# Autodesk Inventor assembly: gearbox
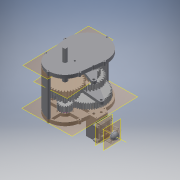
[picture p0: Inventor's stored thumbnail of the model, 180x180]
Saved by Autodesk Inventor 2017 (Build 210142000, 142)
## iProperties
Created: 2018-04-16
Part Number: gearbox
Document SubType Name: Assembly
Designer: RKL
Author: RKL
## Documents named in this file (22)
- C:\Users\RKL\Documents\GitHub\Vane_motor_steam_engine\rotary die grinder engine\transmission\gearbox.iam
- C:\Users\RKL\Documents\GitHub\Vane_motor_steam_engine\rotary die grinder engine\transmission\gearbox\Design Accelerator\Spur Gears1.iam
- C:\Users\RKL\Documents\GitHub\Vane_motor_steam_engine\rotary die grinder engine\transmission\square shaft 1.ipt
- C:\Users\RKL\Documents\GitHub\Vane_motor_steam_engine\rotary die grinder engine\transmission\square bearing adapter.ipt
- C:\Users\RKL\Documents\GitHub\Vane_motor_steam_engine\rotary die grinder engine\transmission\6003 bearing.ipt
- C:\Users\RKL\Documents\GitHub\Vane_motor_steam_engine\rotary die grinder engine\transmission\dog clutch.ipt
- C:\Users\RKL\Documents\GitHub\Vane_motor_steam_engine\rotary die grinder engine\transmission\gearbox\Design Accelerator\Spur Gears2.iam
- C:\Users\RKL\Documents\GitHub\Vane_motor_steam_engine\rotary die grinder engine\transmission\gearbox\Design Accelerator\Spur Gears3.iam
- C:\Users\RKL\Documents\GitHub\Vane_motor_steam_engine\rotary die grinder engine\transmission\gearbox\Design Accelerator\Spur Gears4.iam
- C:\Users\RKL\Documents\GitHub\Vane_motor_steam_engine\rotary die grinder engine\transmission\gearbox\Design Accelerator\Spur Gears5.iam
- C:\Users\RKL\Documents\GitHub\Vane_motor_steam_engine\rotary die grinder engine\transmission\case part 1.ipt
- C:\Users\RKL\Documents\GitHub\Vane_motor_steam_engine\rotary die grinder engine\transmission\fork.ipt
- C:\Users\RKL\Documents\GitHub\Vane_motor_steam_engine\rotary die grinder engine\transmission\shifter box 1.ipt
- C:\Users\RKL\Documents\GitHub\Vane_motor_steam_engine\rotary die grinder engine\transmission\short selector.ipt
- C:\Users\RKL\Documents\GitHub\Vane_motor_steam_engine\rotary die grinder engine\transmission\long selector.ipt
- C:\Users\RKL\Documents\GitHub\Vane_motor_steam_engine\rotary die grinder engine\transmission\shifter cover.ipt
- C:\Users\RKL\Documents\GitHub\Vane_motor_steam_engine\rotary die grinder engine\transmission\shifter cover_MIR.ipt
- C:\Users\RKL\Documents\GitHub\Vane_motor_steam_engine\rotary die grinder engine\transmission\shifter ball.ipt
- C:\Users\RKL\Documents\GitHub\Vane_motor_steam_engine\rotary die grinder engine\transmission\case bottom half.ipt
- C:\Users\RKL\Documents\GitHub\Vane_motor_steam_engine\rotary die grinder engine\transmission\case part 2.ipt
- C:\Users\RKL\Documents\GitHub\Vane_motor_steam_engine\rotary die grinder engine\transmission\case top half.ipt
- C:\Users\RKL\Documents\GitHub\Vane_motor_steam_engine\rotary die grinder engine\transmission\gearbox\gear spacer 1.ipt
## Components (37 placed, 17 different names)
1. Spur Gears:1 [sub-assembly] — Mate:1, Mate:2, Mate:3, Mate:7, Mate:8, Mate:35, Mate:36, Mate:60, Flush:5, Flush:6, Mate:77
2. square shaft 1:1 — Mate:7, Mate:8, Mate:22, Mate:23, Mate:31, Mate:32, Mate:49, Mate:50, Flush:3, Mate:53, Mate:54, Mate:91
3. square shaft 1:2 — Mate:5, Mate:6, Mate:9, Mate:10, Mate:20, Mate:21, Mate:29, Mate:30, Mate:33, Mate:34, Mate:38, Mate:39, Flush:1, Mate:47, Mate:48, Mate:56, Mate:57, Mate:92
4. square bearing adapter:1 — Mate:3, Mate:4, Mate:5, Mate:6
5. 6003 bearing:1 — Mate:1, Mate:2, Mate:4
6. dog clutch:1 — Mate:9, Mate:10, Mate:67, Mate:68
7. Spur Gears:2 [sub-assembly] — Mate:16, Mate:17, Mate:18, Mate:22, Mate:23, Mate:28, Mate:77
8. 6003 bearing:2 — Mate:16, Mate:17, Mate:19
9. square bearing adapter:2 — Mate:18, Mate:19, Mate:20, Mate:21
10. Spur Gears:3 [sub-assembly] — Mate:24, Mate:25, Mate:26, Mate:28, Mate:31, Mate:32, Mate:78, Flush:21, Flush:22
11. 6003 bearing:3 — Mate:24, Mate:25, Mate:27
12. square bearing adapter:3 — Mate:26, Mate:27, Mate:29, Mate:30
13. 6003 bearing:4 — Mate:36, Mate:37, Flush:1, Mate:64
14. square bearing adapter:4 — Mate:33, Mate:34, Mate:35, Mate:37
15. dog clutch:2 — Mate:38, Mate:39, Mate:65, Mate:66
16. Spur Gears:4 [sub-assembly] — Flush:2, Mate:41, Mate:42, Mate:43, Mate:44, Mate:45, Mate:55, Mate:58, Mate:78
17. Spur Gears:5 [sub-assembly] — Flush:2, Mate:41, Mate:49, Mate:50, Mate:51
18. 6003 bearing:5 — Mate:44, Mate:45
19. square bearing adapter:5 — Mate:42, Mate:43, Mate:47, Mate:48
20. 6003 bearing:6 — Mate:58, Mate:59
21. 6003 bearing:7 — Mate:51, Flush:3, Flush:4, Mate:52, Mate:61
22. square bearing adapter:6 — Flush:4, Mate:52, Mate:53, Mate:54
23. square bearing adapter:7 — Mate:55, Mate:56, Mate:57, Mate:59
24. 6003 bearing:8 — Mate:60, Mate:61, Mate:62, Mate:63
25. case part 1:1 — Flush:5, Flush:6, Mate:62, Mate:63, Mate:64, Flush:7, Flush:8, Mate:74, Mate:75, Mate:76, Flush:15, Flush:16, Flush:19, Flush:20, Mate:91, Mate:95, Mate:96
26. fork:1 — Mate:65, Mate:66, Mate:94, Mate:96
27. fork:2 — Mate:67, Mate:68, Mate:93, Mate:95
28. shifter box 1:1 — Flush:7, Flush:8, Flush:9, Flush:10, Mate:71, Mate:72, Mate:73, Mate:74, Mate:75, Mate:76, Flush:11, Flush:12, Mate:80, Mate:81, Mate:82, Flush:13, Flush:14, Mate:84, Mate:85, Mate:86
29. short selector:1 — Flush:9, Flush:10, Mate:71, Mate:72, Mate:73, Mate:94
30. long selector:1 — Flush:11, Flush:12, Mate:80, Mate:81, Mate:82, Mate:93
31. shifter cover:1 — Flush:13, Flush:14, Mate:84, Mate:85, Mate:86, Mate:87, Mate:88, Mate:89, Mate:90
32. shifter cover_MIR:1 — Mate:87, Mate:88, Mate:89
33. shifter ball:1 — Mate:90
34. case bottom half:1 — Flush:15, Flush:16, Flush:17, Flush:18
35. case part 2:1 — Flush:17, Flush:18, Mate:92
36. case top half:1 — Flush:19, Flush:20
37. gear spacer 1:1 — Flush:21, Flush:22
## Relationships (107: Mate 85, Flush 22)
- Mate:1: Spur Gears:1 ↔ 6003 bearing:1
- Mate:2: Spur Gears:1 ↔ 6003 bearing:1
- Mate:3: Spur Gears:1 ↔ square bearing adapter:1
- Mate:4: square bearing adapter:1 ↔ 6003 bearing:1
- Mate:5: square shaft 1:2 ↔ square bearing adapter:1
- Mate:6: square shaft 1:2 ↔ square bearing adapter:1
- Mate:7: Spur Gears:1 ↔ square shaft 1:1
- Mate:8: Spur Gears:1 ↔ square shaft 1:1
- Mate:9: square shaft 1:2 ↔ dog clutch:1
- Mate:10: square shaft 1:2 ↔ dog clutch:1
- Mate:16: Spur Gears:2 ↔ 6003 bearing:2
- Mate:17: Spur Gears:2 ↔ 6003 bearing:2
- Mate:18: Spur Gears:2 ↔ square bearing adapter:2
- Mate:19: 6003 bearing:2 ↔ square bearing adapter:2
- Mate:20: square shaft 1:2 ↔ square bearing adapter:2
- Mate:21: square shaft 1:2 ↔ square bearing adapter:2
- Mate:22: square shaft 1:1 ↔ Spur Gears:2
- Mate:23: square shaft 1:1 ↔ Spur Gears:2
- Mate:24: Spur Gears:3 ↔ 6003 bearing:3
- Mate:25: Spur Gears:3 ↔ 6003 bearing:3
- Mate:26: Spur Gears:3 ↔ square bearing adapter:3
- Mate:27: 6003 bearing:3 ↔ square bearing adapter:3
- Mate:28 (2 mm): Spur Gears:2 ↔ Spur Gears:3
- Mate:29: square shaft 1:2 ↔ square bearing adapter:3
- Mate:30: square shaft 1:2 ↔ square bearing adapter:3
- Mate:31: square shaft 1:1 ↔ Spur Gears:3
- Mate:32: square shaft 1:1 ↔ Spur Gears:3
- Mate:33: square shaft 1:2 ↔ square bearing adapter:4
- Mate:34: square shaft 1:2 ↔ square bearing adapter:4
- Mate:35: Spur Gears:1 ↔ square bearing adapter:4
- Mate:36: Spur Gears:1 ↔ 6003 bearing:4
- Mate:37: 6003 bearing:4 ↔ square bearing adapter:4
- Mate:38: square shaft 1:2 ↔ dog clutch:2
- Mate:39: square shaft 1:2 ↔ dog clutch:2
- Flush:1: square shaft 1:2 ↔ 6003 bearing:4
- Flush:2: Spur Gears:4 ↔ Spur Gears:5
- Mate:41 (25 mm): Spur Gears:4 ↔ Spur Gears:5
- Mate:42: Spur Gears:4 ↔ square bearing adapter:5
- Mate:43: Spur Gears:4 ↔ square bearing adapter:5
- Mate:44: Spur Gears:4 ↔ 6003 bearing:5
- Mate:45: Spur Gears:4 ↔ 6003 bearing:5
- Mate:47: square shaft 1:2 ↔ square bearing adapter:5
- Mate:48: square shaft 1:2 ↔ square bearing adapter:5
- Mate:49: square shaft 1:1 ↔ Spur Gears:5
- Mate:50: square shaft 1:1 ↔ Spur Gears:5
- Mate:51: Spur Gears:5 ↔ 6003 bearing:7
- Flush:3: square shaft 1:1 ↔ 6003 bearing:7
- Flush:4: 6003 bearing:7 ↔ square bearing adapter:6
- Mate:52: 6003 bearing:7 ↔ square bearing adapter:6
- Mate:53: square shaft 1:1 ↔ square bearing adapter:6
- Mate:54: square shaft 1:1 ↔ square bearing adapter:6
- Mate:55: Spur Gears:4 ↔ square bearing adapter:7
- Mate:56: square shaft 1:2 ↔ square bearing adapter:7
- Mate:57: square shaft 1:2 ↔ square bearing adapter:7
- Mate:58: Spur Gears:4 ↔ 6003 bearing:6
- Mate:59: 6003 bearing:6 ↔ square bearing adapter:7
- Mate:60: Spur Gears:1 ↔ 6003 bearing:8
- Mate:61: 6003 bearing:7 ↔ 6003 bearing:8
- Flush:5: Spur Gears:1 ↔ case part 1:1
- Flush:6: Spur Gears:1 ↔ case part 1:1
- Mate:62: 6003 bearing:8 ↔ case part 1:1
- Mate:63: 6003 bearing:8 ↔ case part 1:1
- Mate:64: 6003 bearing:4 ↔ case part 1:1
- Mate:65: dog clutch:2 ↔ fork:1
- Mate:66: dog clutch:2 ↔ fork:1
- Mate:67: dog clutch:1 ↔ fork:2
- Mate:68: dog clutch:1 ↔ fork:2
- Flush:7: case part 1:1 ↔ shifter box 1:1
- Flush:8: case part 1:1 ↔ shifter box 1:1
- Flush:9: shifter box 1:1 ↔ short selector:1
- Flush:10: shifter box 1:1 ↔ short selector:1
- Mate:71: shifter box 1:1 ↔ short selector:1
- Mate:72: shifter box 1:1 ↔ short selector:1
- Mate:73 (16 mm): shifter box 1:1 ↔ short selector:1
- Mate:74: case part 1:1 ↔ shifter box 1:1
- Mate:75: case part 1:1 ↔ shifter box 1:1
- Mate:76: case part 1:1 ↔ shifter box 1:1
- Mate:77 (26 mm): Spur Gears:1 ↔ Spur Gears:2
- Mate:78 (26 mm): Spur Gears:3 ↔ Spur Gears:4
- Flush:11: shifter box 1:1 ↔ long selector:1
- Flush:12: shifter box 1:1 ↔ long selector:1
- Mate:80: shifter box 1:1 ↔ long selector:1
- Mate:81: shifter box 1:1 ↔ long selector:1
- Mate:82 (16 mm): shifter box 1:1 ↔ long selector:1
- Flush:13: shifter box 1:1 ↔ shifter cover:1
- Flush:14: shifter box 1:1 ↔ shifter cover:1
- Mate:84: shifter box 1:1 ↔ shifter cover:1
- Mate:85: shifter box 1:1 ↔ shifter cover:1
- Mate:86: shifter box 1:1 ↔ shifter cover:1
- Mate:87: shifter cover:1 ↔ shifter cover_MIR:1
- Mate:88: shifter cover:1 ↔ shifter cover_MIR:1
- Mate:89: shifter cover:1 ↔ shifter cover_MIR:1
- Mate:90: shifter cover:1 ↔ shifter ball:1
- Flush:15: case part 1:1 ↔ case bottom half:1
- Flush:16: case part 1:1 ↔ case bottom half:1
- Flush:17: case bottom half:1 ↔ case part 2:1
- Flush:18: case bottom half:1 ↔ case part 2:1
- Flush:19: case part 1:1 ↔ case top half:1
- Flush:20: case part 1:1 ↔ case top half:1
- Mate:91: square shaft 1:1 ↔ case part 1:1
- Mate:92: square shaft 1:2 ↔ case part 2:1
- Mate:93 (61.5 mm): fork:2 ↔ long selector:1
- Mate:94 (129.5 mm): fork:1 ↔ short selector:1
- Mate:95: case part 1:1 ↔ fork:2
- Mate:96: case part 1:1 ↔ fork:1
- Flush:21: Spur Gears:3 ↔ gear spacer 1:1
- Flush:22: Spur Gears:3 ↔ gear spacer 1:1
